# Autodesk Inventor assembly: TFT35 Mount
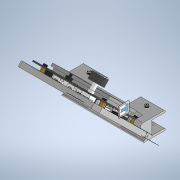
[picture p0: Inventor's stored thumbnail of the model, 180x180]
Saved by Autodesk Inventor 2022 (Build 260153000, 153)
## iProperties
Created: 2022-04-02
Part Number: TFT35 Mount
Document SubType Name: Assembly
Designer: Nick
Author: Nick
## Documents named in this file (9)
- Y:\Projects\Bibble0\SubAsm\TFT35 Mount.iam
- Y:\Projects\Bibble0\Electronics\TFT35.ipt
- Y:\Projects\Bibble0\3D printed\LCD Mount 1.ipt
- Y:\Projects\Bibble0\Hardware\6mm x 6mm Magnet.ipt
- Y:\Projects\Bibble0\Hardware\5mm M3 Brass Standoff.ipt
- Y:\Projects\Bibble0\Hardware\M3 x 4 mm SHCS.ipt
- Y:\Projects\Bibble0\3D printed\LCD Mount 2 HSI.iam
- Y:\Projects\Bibble0\Hardware\M3 x 6 mm SHCS.ipt
- Y:\Projects\Bibble0\Hardware\M3 T-Slot Nut.ipt
## Components (23 placed, 8 different names)
1. TFT35:1 — Insert:11, Insert:12, Insert:13, Insert:14, Insert:20, Insert:21
2. LCD Mount 1:1 — Insert:2, Insert:3, Insert:24, Insert:25, Angle:1, Insert:26, Insert:27, Insert:28, Insert:29, Insert:30, Insert:31, Insert:32, Angle:5
3. LCD Mount 2 HSI:1 [sub-assembly] — Insert:16, Insert:17, Insert:18, Insert:19, Insert:22, Insert:23, Insert:32, Angle:5
4. 6mm x 6mm Magnet:1 — Insert:2
5. 6mm x 6mm Magnet:2 — Insert:3
6. 6mm x 6mm Magnet:3 — Insert:23
7. 6mm x 6mm Magnet:4 — Insert:22
8. 5mm M3 Brass Standoff:1 — Insert:18
9. 5mm M3 Brass Standoff:2 — Insert:16, Insert:20
10. 5mm M3 Brass Standoff:3 — Insert:17
11. 5mm M3 Brass Standoff:4 — Insert:19, Insert:21
12. M3 x 4 mm SHCS:1 — Insert:11
13. M3 x 4 mm SHCS:2 — Insert:14
14. M3 x 4 mm SHCS:3 — Insert:12
15. M3 x 4 mm SHCS:4 — Insert:13
16. M3 x 6 mm SHCS:1 — Insert:24
17. M3 T-Slot Nut:1 — Insert:25, Angle:1, Angle:2, Angle:3, Angle:4
18. M3 x 6 mm SHCS:2 — Insert:26
19. M3 x 6 mm SHCS:3 — Insert:28
20. M3 x 6 mm SHCS:4 — Insert:27
21. M3 T-Slot Nut:2 — Insert:29, Angle:3
22. M3 T-Slot Nut:3 — Insert:30, Angle:4
23. M3 T-Slot Nut:4 — Insert:31, Angle:2
## Relationships (28: Insert 23, Angle 5)
- Insert:2: LCD Mount 1:1 ↔ 6mm x 6mm Magnet:1
- Insert:3: LCD Mount 1:1 ↔ 6mm x 6mm Magnet:2
- Insert:11: TFT35:1 ↔ M3 x 4 mm SHCS:1
- Insert:12: TFT35:1 ↔ M3 x 4 mm SHCS:3
- Insert:13: TFT35:1 ↔ M3 x 4 mm SHCS:4
- Insert:14: TFT35:1 ↔ M3 x 4 mm SHCS:2
- Insert:16: LCD Mount 2 HSI:1 ↔ 5mm M3 Brass Standoff:2
- Insert:17: LCD Mount 2 HSI:1 ↔ 5mm M3 Brass Standoff:3
- Insert:18: LCD Mount 2 HSI:1 ↔ 5mm M3 Brass Standoff:1
- Insert:19: LCD Mount 2 HSI:1 ↔ 5mm M3 Brass Standoff:4
- Insert:20: TFT35:1 ↔ 5mm M3 Brass Standoff:2
- Insert:21: TFT35:1 ↔ 5mm M3 Brass Standoff:4
- Insert:22: LCD Mount 2 HSI:1 ↔ 6mm x 6mm Magnet:4
- Insert:23: LCD Mount 2 HSI:1 ↔ 6mm x 6mm Magnet:3
- Insert:24: LCD Mount 1:1 ↔ M3 x 6 mm SHCS:1
- Insert:25: LCD Mount 1:1 ↔ M3 T-Slot Nut:1
- Angle:1 (0 deg): LCD Mount 1:1 ↔ M3 T-Slot Nut:1
- Insert:26: LCD Mount 1:1 ↔ M3 x 6 mm SHCS:2
- Insert:27: LCD Mount 1:1 ↔ M3 x 6 mm SHCS:4
- Insert:28: LCD Mount 1:1 ↔ M3 x 6 mm SHCS:3
- Insert:29: LCD Mount 1:1 ↔ M3 T-Slot Nut:2
- Insert:30: LCD Mount 1:1 ↔ M3 T-Slot Nut:3
- Insert:31: LCD Mount 1:1 ↔ M3 T-Slot Nut:4
- Angle:2 (0 deg): M3 T-Slot Nut:1 ↔ M3 T-Slot Nut:4
- Angle:3 (0 deg): M3 T-Slot Nut:1 ↔ M3 T-Slot Nut:2
- Angle:4 (0 deg): M3 T-Slot Nut:1 ↔ M3 T-Slot Nut:3
- Insert:32: LCD Mount 1:1 ↔ LCD Mount 2 HSI:1
- Angle:5 (0 deg): LCD Mount 1:1 ↔ LCD Mount 2 HSI:1
